# Autodesk Inventor assembly: Gesamtbaugruppe
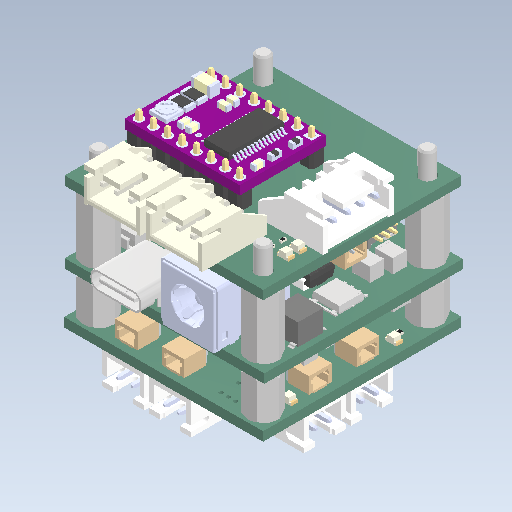
[picture p0: Inventor's stored thumbnail of the model, 512x512]
Saved by Autodesk Inventor 2025 (Build 290162010, 162A)
## iProperties
Created: 2025-03-12
Part Number: Gesamtbaugruppe
Document SubType Name: Assembly
Designer: jan
Author: jan
## Documents named in this file (4)
- C:\Users\jan\Documents\github\fiberprinter-electronics\2nd-mainboard-pcb\cadv2\Gesamtbaugruppe.iam
- C:\Users\jan\Documents\github\fiberprinter-electronics\2nd-mainboard-pcb\cadv2\Leistung\ExportV2.iam
- C:\Users\jan\Documents\github\fiberprinter-electronics\2nd-mainboard-pcb\cadv2\Fans\ExportV2.iam
- C:\Users\jan\Documents\github\fiberprinter-electronics\2nd-mainboard-pcb\cadv2\Motoren\ExportV2.iam
## Components (3 placed, 1 different names)
1. ExportV2:1 [sub-assembly] — Passend:1, Passend:2, Passend:3, Passend:4, Passend:5, Passend:6
2. ExportV2:2 [sub-assembly] — Passend:1, Passend:2, Passend:3
3. ExportV2:3 [sub-assembly] — Passend:4, Passend:5, Passend:6
## Relationships (6: Mate 6)
- Passend:1 [Mate]: ExportV2:1 ↔ ExportV2:2
- Passend:2 [Mate]: ExportV2:1 ↔ ExportV2:2
- Passend:3 [Mate]: ExportV2:1 ↔ ExportV2:2
- Passend:4 [Mate]: ExportV2:1 ↔ ExportV2:3
- Passend:5 [Mate]: ExportV2:1 ↔ ExportV2:3
- Passend:6 [Mate]: ExportV2:1 ↔ ExportV2:3
